# Autodesk Inventor assembly: Sampling Connections
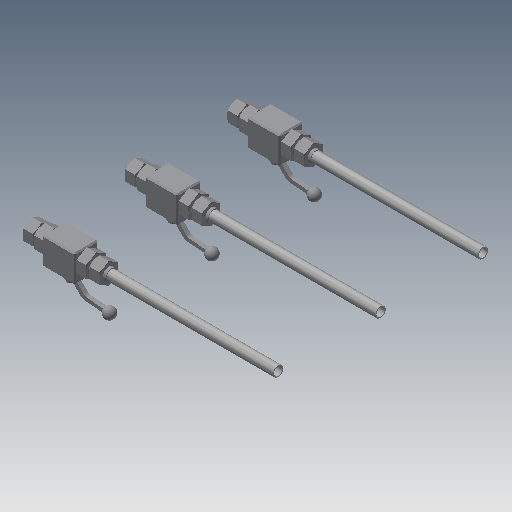
[picture p0: Inventor's stored thumbnail of the model, 512x512]
Saved by Autodesk Inventor 2020 (Build 240152000, 152)
## iProperties
Created: 2009-08-10
Part Number: Sampling Connections
Document SubType Name: Assembly
Designer: Demir Ali
Description: Sampling Connections
Stock Number: NA
Author: Demir Ali
Title: In House Assembly
Revision Number: A
## Documents named in this file (3)
- C:\Users\hallc\Desktop\Process Equipment\Workspace\Options\Sampling Connections.iam
- C:\Users\hallc\Desktop\Process Equipment\Workspace\Supplier Content\Valves\BO_KHV__15_L_NW__13_WAL602203__offen_.ipt
- C:\Users\hallc\Desktop\Process Equipment\Workspace\Components\DIN 2462 Tube 15 x 1.5 - 250.ipt
## Components (6 placed, 2 different names)
1. BO-KHV  15 L/NW  13 WAL602203 (offen):1 — Insert:1, Angle:1
2. DIN 2462 Tube 15 x 1.5 - 250:1 — Insert:1
3. BO-KHV  15 L/NW  13 WAL602203 (offen):2
4. DIN 2462 Tube 15 x 1.5 - 250:2
5. BO-KHV  15 L/NW  13 WAL602203 (offen):3
6. DIN 2462 Tube 15 x 1.5 - 250:3
## Component patterns: (3 elements, first: BO-KHV  15 L/NW  13 WAL602203 (offen):1 + DIN 2462 Tube 15 x 1.5 - 250:1)
## Relationships (2: Insert 1, Angle 1)
- Insert:1: BO-KHV  15 L/NW  13 WAL602203 (offen):1 ↔ DIN 2462 Tube 15 x 1.5 - 250:1
- Angle:1 (0 deg): BO-KHV  15 L/NW  13 WAL602203 (offen):1
